# Autodesk Inventor assembly: KB33-046-002 - Привод в сборе
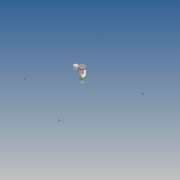
[picture p0: Inventor's stored thumbnail of the model, 180x180]
Saved by Autodesk Inventor 2020 (Build 240168000, 168)
## iProperties
Created: 2021-06-21
Part Number: KB33-046-002 - Привод в сборе
Document SubType Name: Assembly
Designer: Петров Иван
Mass: 1234.32 g
Surface Area: 1916.85 cm^2
Volume: 1228.13 cm^3
Density: 1.00504 g/cm^3
Author: Петров Иван
## Documents named in this file (11)
- C:\Users\Ivan\Documents\GitHub\RoboPatrol\design\KB33-046-002 - Привод в сборе.iam
- C:\Users\Ivan\Documents\GitHub\RoboPatrol\design\KB33-046-002-001 - Крепление.ipt
- C:\Users\Ivan\Documents\GitHub\RoboPatrol\design\standart_components\dc_gear_motor_12V_500rpm\dc_gear_motor_12V_500rpm.ipt
- C:\Users\Ivan\Documents\GitHub\RoboPatrol\design\standart_components\WheelBig\колесо большое1.iam
- C:\Users\Ivan\Documents\GitHub\RoboPatrol\design\KB33-046-002-002 - Втулка.ipt
- C:\Users\Ivan\Documents\GitHub\RoboPatrol\design\KB33-046-002-003 - Фиксирующая гайка.ipt
- C:\Users\Ivan\Documents\GitHub\RoboPatrol\design\KB33-046-002-004 - Колесо энкодера.ipt
- C:\Users\Ivan\Documents\GitHub\RoboPatrol\design\standart_components\Standart optical endstop.ipt
- C:\Users\Ivan\Documents\GitHub\RoboPatrol\design\KB33-046-002-005 - Кожух датчика.ipt
- C:\Users\Ivan\Documents\GitHub\RoboPatrol\design\KB33-046-002-006 - Заглушка.ipt
- C:\Users\Ivan\Documents\GitHub\RoboPatrol\design\KB33-046-002-007 - Крышка мотора.ipt
## Components (12 placed, 10 different names)
1. KB33-046-002-001 - Крепление:1 — Заподлицо:1, Совмещение:1, Совмещение:2, Угол:6, Совмещение:17, Совмещение:19, Совмещение:24, Совмещение:25, Совмещение:26
2. dc_gear_motor_12V_500rpm:1 — Заподлицо:1, Совмещение:1, Совмещение:2, Совмещение:3, Совмещение:4, Совмещение:5, Совмещение:6, Угол:1
3. колесо большое1:1 [sub-assembly] — Совмещение:3, Совмещение:4, Угол:2, Совмещение:8, Совмещение:10
4. KB33-046-002-002 - Втулка:1 — Совмещение:5, Совмещение:6, Угол:1, Совмещение:7, Совмещение:9, Совмещение:11, Угол:3, Совмещение:12, Совмещение:16, Совмещение:18, Совмещение:20
5. KB33-046-002-003 - Фиксирующая гайка:1 — Совмещение:7, Угол:2, Совмещение:8, Угол:4
6. KB33-046-002-003 - Фиксирующая гайка:2 — Совмещение:9, Совмещение:10, Угол:4
7. KB33-046-002-003 - Фиксирующая гайка:3 — Совмещение:11, Угол:3, Совмещение:12, Угол:5, Заподлицо:2
8. KB33-046-002-004 - Колесо энкодера:1 — Угол:5, Касательность:1, Совмещение:15, Совмещение:20, Заподлицо:2
9. Standart optical endstop:1 — Касательность:1, Угол:6, Совмещение:15, Совмещение:16, Совмещение:21
10. KB33-046-002-005 - Кожух датчика:1 — Совмещение:17, Совмещение:18, Совмещение:19, Совмещение:22, Совмещение:23
11. KB33-046-002-006 - Заглушка:1 — Совмещение:21, Совмещение:22, Совмещение:23
12. KB33-046-002-007 - Крышка мотора:1 — Совмещение:24, Совмещение:25, Совмещение:26
## Relationships (33: Mate 24, Angle 6, Flush 2, Tangent 1)
- Заподлицо:1 [Flush]: KB33-046-002-001 - Крепление:1 ↔ dc_gear_motor_12V_500rpm:1
- Совмещение:1 [Mate]: KB33-046-002-001 - Крепление:1 ↔ dc_gear_motor_12V_500rpm:1
- Совмещение:2 [Mate]: KB33-046-002-001 - Крепление:1 ↔ dc_gear_motor_12V_500rpm:1
- Совмещение:3 [Mate] (30 mm): dc_gear_motor_12V_500rpm:1 ↔ колесо большое1:1
- Совмещение:4 [Mate]: dc_gear_motor_12V_500rpm:1 ↔ колесо большое1:1
- Совмещение:5 [Mate]: dc_gear_motor_12V_500rpm:1 ↔ KB33-046-002-002 - Втулка:1
- Совмещение:6 [Mate]: dc_gear_motor_12V_500rpm:1 ↔ KB33-046-002-002 - Втулка:1
- Угол:1 [Angle] (180 deg): dc_gear_motor_12V_500rpm:1 ↔ KB33-046-002-002 - Втулка:1
- Совмещение:7 [Mate]: KB33-046-002-002 - Втулка:1 ↔ KB33-046-002-003 - Фиксирующая гайка:1
- Угол:2 [Angle] (0 deg): колесо большое1:1 ↔ KB33-046-002-003 - Фиксирующая гайка:1
- Совмещение:8 [Mate]: колесо большое1:1 ↔ KB33-046-002-003 - Фиксирующая гайка:1
- Совмещение:9 [Mate]: KB33-046-002-002 - Втулка:1 ↔ KB33-046-002-003 - Фиксирующая гайка:2
- Совмещение:10 [Mate]: колесо большое1:1 ↔ KB33-046-002-003 - Фиксирующая гайка:2
- Совмещение:11 [Mate]: KB33-046-002-002 - Втулка:1 ↔ KB33-046-002-003 - Фиксирующая гайка:3
- Угол:3 [Angle] (0 deg): KB33-046-002-002 - Втулка:1 ↔ KB33-046-002-003 - Фиксирующая гайка:3
- Совмещение:12 [Mate]: KB33-046-002-002 - Втулка:1 ↔ KB33-046-002-003 - Фиксирующая гайка:3
- Угол:4 [Angle] (0 deg): KB33-046-002-003 - Фиксирующая гайка:1 ↔ KB33-046-002-003 - Фиксирующая гайка:2
- Угол:5 [Angle] (0 deg): KB33-046-002-003 - Фиксирующая гайка:3 ↔ KB33-046-002-004 - Колесо энкодера:1
- Касательность:1 [Tangent] (2.5 mm): KB33-046-002-004 - Колесо энкодера:1 ↔ Standart optical endstop:1
- Угол:6 [Angle] (250 deg): KB33-046-002-001 - Крепление:1 ↔ Standart optical endstop:1
- Совмещение:15 [Mate] (1 mm): KB33-046-002-004 - Колесо энкодера:1 ↔ Standart optical endstop:1
- Совмещение:16 [Mate] (-4 mm): KB33-046-002-002 - Втулка:1 ↔ Standart optical endstop:1
- Совмещение:17 [Mate]: KB33-046-002-001 - Крепление:1 ↔ KB33-046-002-005 - Кожух датчика:1
- Совмещение:18 [Mate]: KB33-046-002-002 - Втулка:1 ↔ KB33-046-002-005 - Кожух датчика:1
- Совмещение:19 [Mate]: KB33-046-002-001 - Крепление:1 ↔ KB33-046-002-005 - Кожух датчика:1
- Совмещение:20 [Mate]: KB33-046-002-002 - Втулка:1 ↔ KB33-046-002-004 - Колесо энкодера:1
- Заподлицо:2 [Flush]: KB33-046-002-003 - Фиксирующая гайка:3 ↔ KB33-046-002-004 - Колесо энкодера:1
- Совмещение:21 [Mate]: Standart optical endstop:1 ↔ KB33-046-002-006 - Заглушка:1
- Совмещение:22 [Mate]: KB33-046-002-005 - Кожух датчика:1 ↔ KB33-046-002-006 - Заглушка:1
- Совмещение:23 [Mate]: KB33-046-002-005 - Кожух датчика:1 ↔ KB33-046-002-006 - Заглушка:1
- Совмещение:24 [Mate]: KB33-046-002-001 - Крепление:1 ↔ KB33-046-002-007 - Крышка мотора:1
- Совмещение:25 [Mate]: KB33-046-002-001 - Крепление:1 ↔ KB33-046-002-007 - Крышка мотора:1
- Совмещение:26 [Mate]: KB33-046-002-001 - Крепление:1 ↔ KB33-046-002-007 - Крышка мотора:1
